# Autodesk Inventor assembly: Ring Funnel
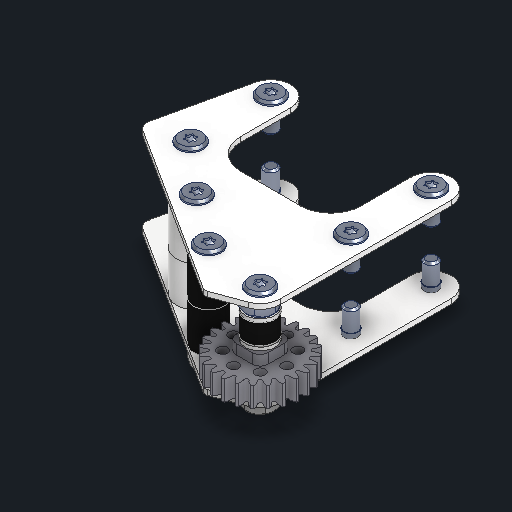
[picture p0: Inventor's stored thumbnail of the model, 512x512]
Saved by Autodesk Inventor 2025.1 (Build 291241000, 241)
## iProperties
Created: 2024-11-11
Part Number: Ring Funnel
Document SubType Name: Assembly
Designer: avere
Author: avere
## Documents named in this file (18)
- C:\Users\avere\VEX\High Stakes\CAD\V3\Chassis\Drivebay Left\Ring Funnel.iam
- C:\Users\avere\VEX\High Stakes\CAD\V3\Chassis\Drivebay Left\Custom Parts\Funnel Gusset.ipt
- C:\Users\avere\VEX\High Stakes\CAD\ROBOPROS-CAD-Inventor\Motion\Spacers\Spacer Nylon .375 OD\NSpacer .375 OD x .500.ipt
- C:\Users\avere\VEX\High Stakes\CAD\ROBOPROS-CAD-Inventor\Motion\Spacers\Spacer Nylon .375 OD.ipt
- C:\Users\avere\VEX\High Stakes\CAD\ROBOPROS-CAD-Inventor\Motion\Spacers\Spacer Nylon .500 OD\NSpacer White .500 OD x .500.ipt
- C:\Users\avere\VEX\High Stakes\CAD\ROBOPROS-CAD-Inventor\Motion\Spacers\Spacer Nylon .500 OD.ipt
- C:\Users\avere\VEX\High Stakes\CAD\ROBOPROS-CAD-Inventor\Modified Parts\Half Cut HS 24T Gear, No Insert.ipt
- C:\Users\avere\VEX\High Stakes\CAD\ROBOPROS-CAD-Inventor\Structure\Hardware\Nut Keps.ipt
- C:\Users\avere\VEX\High Stakes\CAD\ROBOPROS-CAD-Inventor\Motion\Spacers\Spacer Nylon .375 OD\NSpacer .375 OD x .250.ipt
- C:\Users\avere\VEX\High Stakes\CAD\ROBOPROS-CAD-Inventor\Motion\Spacers\Washer Teflon\TWasher .375 OD x .04000.ipt
- C:\Users\avere\VEX\High Stakes\CAD\ROBOPROS-CAD-Inventor\Motion\Spacers\Washer Teflon.ipt
- C:\Users\avere\VEX\High Stakes\CAD\ROBOPROS-CAD-Inventor\Motion\Spacers\Washer Steel\SWasher .375 OD x .015625.ipt
- C:\Users\avere\VEX\High Stakes\CAD\ROBOPROS-CAD-Inventor\Motion\Spacers\Washer Steel.ipt
- C:\Users\avere\VEX\High Stakes\CAD\ROBOPROS-CAD-Inventor\Structure\Hardware\Screw Steel - Star\SScrew Star Smooth 1.250.ipt
- C:\Users\avere\VEX\High Stakes\CAD\ROBOPROS-CAD-Inventor\Structure\Hardware\Screw Steel - Star.ipt
- C:\Users\avere\VEX\High Stakes\CAD\ROBOPROS-CAD-Inventor\Structure\Hardware\Nut Nylon Thread-Forming.ipt
- C:\Users\avere\VEX\High Stakes\CAD\ROBOPROS-CAD-Inventor\Structure\Hardware\Screw Shoulder Robosource\SScrew Shoulder Smooth .375 x .12.ipt
- C:\Users\avere\VEX\High Stakes\CAD\ROBOPROS-CAD-Inventor\Structure\Hardware\Screw Shoulder Robosource.ipt
## Components (26 placed, 11 different names)
1. Funnel Gusset:1 — Insert:4, Insert:6, Insert:17, Insert:18, Insert:19, Insert:20
2. Funnel Gusset:2 — Insert:7, Mate:1, Insert:12, Insert:13, Insert:15, Insert:16, Insert:21
3. NSpacer .375 OD x .500:2 — Insert:2, Mate:1
4. NSpacer .375 OD x .500:4 — Insert:2, Insert:4
5. NSpacer White .500 OD x .500:1 — Insert:5, Insert:6
6. NSpacer White .500 OD x .500:2 — Insert:5, Insert:7
7. Half Cut HS 24T Gear, No Insert:1
8. Nut Keps:1 — Insert:13, Insert:14
9. NSpacer .375 OD x .250:5
10. TWasher .375 OD x .04000:1
11. TWasher .375 OD x .04000:2 — Insert:14
12. SWasher .375 OD x .015625:1
13. SScrew Star Smooth 1.250:1 — Insert:12
14. SScrew Star Smooth 1.250:2 — Insert:15
15. SScrew Star Smooth 1.250:3 — Insert:16
16. Nut Nylon Thread-Forming:1 — Insert:19
17. Nut Nylon Thread-Forming:2 — Insert:18
18. Nut Nylon Thread-Forming:3 — Insert:17
19. SScrew Shoulder Smooth .375 x .12:1 — Insert:20
20. SScrew Shoulder Smooth .375 x .12:2
21. SScrew Shoulder Smooth .375 x .12:3
22. SScrew Shoulder Smooth .375 x .12:4
23. SScrew Shoulder Smooth .375 x .12:5 — Insert:21
24. SScrew Shoulder Smooth .375 x .12:6
25. SScrew Shoulder Smooth .375 x .12:7
26. SScrew Shoulder Smooth .375 x .12:8
## Component patterns: Bottom Boxing Screws (4 elements), Top Boxing Screws (4 elements)
## Relationships (20: Insert 19, Mate 1)
- Insert:2: NSpacer .375 OD x .500:2 ↔ NSpacer .375 OD x .500:4
- Insert:4: Funnel Gusset:1 ↔ NSpacer .375 OD x .500:4
- Insert:5: NSpacer White .500 OD x .500:1 ↔ NSpacer White .500 OD x .500:2
- Insert:6: Funnel Gusset:1 ↔ NSpacer White .500 OD x .500:1
- Insert:7: Funnel Gusset:2 ↔ NSpacer White .500 OD x .500:2
- Mate:1: Funnel Gusset:2 ↔ NSpacer .375 OD x .500:2
- [Insert]: NSpacer .375 OD x .250:5 ↔ TWasher .375 OD x .04000:2
- [Insert]: NSpacer .375 OD x .250:5 ↔ SWasher .375 OD x .015625:1
- [Insert]: TWasher .375 OD x .04000:1 ↔ SWasher .375 OD x .015625:1
- [Insert]: Half Cut HS 24T Gear, No Insert:1 ↔ TWasher .375 OD x .04000:1
- Insert:12: Funnel Gusset:2 ↔ SScrew Star Smooth 1.250:1
- Insert:13: Funnel Gusset:2 ↔ Nut Keps:1
- Insert:14: Nut Keps:1 ↔ TWasher .375 OD x .04000:2
- Insert:15: Funnel Gusset:2 ↔ SScrew Star Smooth 1.250:2
- Insert:16: Funnel Gusset:2 ↔ SScrew Star Smooth 1.250:3
- Insert:17: Funnel Gusset:1 ↔ Nut Nylon Thread-Forming:3
- Insert:18: Funnel Gusset:1 ↔ Nut Nylon Thread-Forming:2
- Insert:19: Funnel Gusset:1 ↔ Nut Nylon Thread-Forming:1
- Insert:20: Funnel Gusset:1 ↔ SScrew Shoulder Smooth .375 x .12:1
- Insert:21: Funnel Gusset:2 ↔ SScrew Shoulder Smooth .375 x .12:5
